# Autodesk Inventor assembly: SplitterBlock
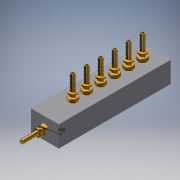
[picture p0: Inventor's stored thumbnail of the model, 180x180]
Saved by Autodesk Inventor 2018 (Build 220112000, 112)
## iProperties
Created: 2020-03-29
Part Number: SplitterBlock
Document SubType Name: Assembly
Designer: emile
Author: emile
## Documents named in this file (3)
- C:\Users\emile\OneDrive\Documents\GitHub\VentilatorCovid19\Respirator\MultiLine\SplitterBlock.iam
- C:\Users\emile\OneDrive\Documents\GitHub\VentilatorCovid19\Respirator\Peep\AirPressure\Splitter.ipt
- C:\Users\emile\OneDrive\Documents\GitHub\VentilatorCovid19\Respirator\Peep\AirPressure\Brass Barbed Hose Fitting for Air and Water.ipt
## Components (8 placed, 2 different names)
1. Splitter:1 — Mate:1, Mate:2, Mate:3, Mate:4
2. Brass Barbed Hose Fitting for Air and Water:7 — Mate:3, Mate:4
3. Brass Barbed Hose Fitting for Air and Water:1 — Mate:1, Mate:2
4. Brass Barbed Hose Fitting for Air and Water:2
5. Brass Barbed Hose Fitting for Air and Water:3
6. Brass Barbed Hose Fitting for Air and Water:4
7. Brass Barbed Hose Fitting for Air and Water:5
8. Brass Barbed Hose Fitting for Air and Water:6
## Component patterns: (6 elements, first: Brass Barbed Hose Fitting for Air and Water:1)
## Relationships (4: Mate 4)
- Mate:1: Splitter:1 ↔ Brass Barbed Hose Fitting for Air and Water:1
- Mate:2: Splitter:1 ↔ Brass Barbed Hose Fitting for Air and Water:1
- Mate:3: Splitter:1 ↔ Brass Barbed Hose Fitting for Air and Water:7
- Mate:4: Splitter:1 ↔ Brass Barbed Hose Fitting for Air and Water:7
